# Autodesk Inventor assembly: cortador
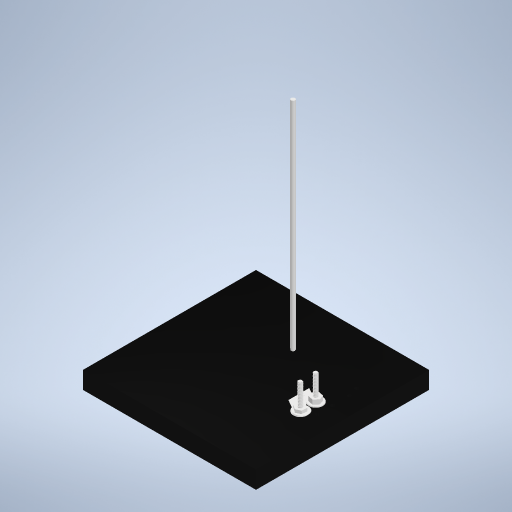
[picture p0: Inventor's stored thumbnail of the model, 512x512]
Saved by Autodesk Inventor 2024.3 (Build 283343000, 343)
## iProperties
Created: 2025-01-13
Part Number: cortador
Document SubType Name: Assembly
Designer: AdminForWorker
Title: cortador v2
Author: AdminForWorker
## Documents named in this file (7)
- C:\Users\leivi\OneDrive\Documentos\GitHub\Practica-1-Ensamble\ensamble cortardora\cortador.iam
- C:\Users\leivi\OneDrive\Documentos\GitHub\Practica-1-Ensamble\ensamble cortardora\base.ipt
- C:\Users\leivi\OneDrive\Documentos\GitHub\Practica-1-Ensamble\ensamble cortardora\tornillo.ipt
- C:\Users\leivi\OneDrive\Documentos\GitHub\Practica-1-Ensamble\ensamble cortardora\tuerca.ipt
- C:\Users\leivi\OneDrive\Documentos\GitHub\Practica-1-Ensamble\ensamble cortardora\golilla.ipt
- C:\Users\leivi\OneDrive\Documentos\GitHub\Practica-1-Ensamble\ensamble cortardora\cuchilla.ipt
- C:\Users\leivi\OneDrive\Documentos\GitHub\Practica-1-Ensamble\ensamble cortardora\varilla.ipt
## Components (14 placed, 6 different names)
1. base:1 — Coincidencia:14
2. tornillo:1 — Coincidencia:9, Coincidencia:11, Coincidencia:13, Coincidencia:14
3. tuerca:1 — Coincidencia:7, Coincidencia:8
4. golilla:1 — Coincidencia:9, Coincidencia:10, Coincidencia:12
5. cuchilla:1 — Coincidencia:1, Coincidencia:2, Coincidencia:10
6. tornillo:3 — Coincidencia:4, Coincidencia:5, Coincidencia:7
7. varilla:1
8. golilla:2 — Coincidencia:11
9. golilla:4 — Coincidencia:1
10. golilla:6 — Coincidencia:6
11. golilla:7 — Coincidencia:2, Coincidencia:3, Coincidencia:5, Coincidencia:6
12. golilla:9 — Coincidencia:12
13. golilla:10 — Coincidencia:3, Coincidencia:4, Coincidencia:8
14. tuerca:2 — Coincidencia:13
## Relationships (14: Mate 14)
- Coincidencia:1 [Mate]: cuchilla:1 ↔ golilla:4
- Coincidencia:2 [Mate]: cuchilla:1 ↔ golilla:7
- Coincidencia:3 [Mate]: golilla:7 ↔ golilla:10
- Coincidencia:4 [Mate]: tornillo:3 ↔ golilla:10
- Coincidencia:5 [Mate]: tornillo:3 ↔ golilla:7
- Coincidencia:6 [Mate]: golilla:6 ↔ golilla:7
- Coincidencia:7 [Mate]: tuerca:1 ↔ tornillo:3
- Coincidencia:8 [Mate]: tuerca:1 ↔ golilla:10
- Coincidencia:9 [Mate]: tornillo:1 ↔ golilla:1
- Coincidencia:10 [Mate]: golilla:1 ↔ cuchilla:1
- Coincidencia:11 [Mate]: tornillo:1 ↔ golilla:2
- Coincidencia:12 [Mate]: golilla:1 ↔ golilla:9
- Coincidencia:13 [Mate]: tornillo:1 ↔ tuerca:2
- Coincidencia:14 [Mate]: base:1 ↔ tornillo:1
